# Autodesk Inventor assembly: Counter2
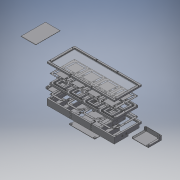
[picture p0: Inventor's stored thumbnail of the model, 180x180]
Saved by Autodesk Inventor 2016 SP2 (Build 200236200, 236)
## iProperties
Created: 2018-06-10
Part Number: Counter2
Material: Generisch
Document SubType Name: Assembly
Designer: Nils
Author: Nils
## Documents named in this file (17)
- C:\Users\Nils\Documents\Inventor\Bastelleien\Counter\Counter2.iam
- C:\Users\Nils\Documents\Inventor\Bastelleien\Counter\Segment_V4.ipt
- C:\Users\Nils\Documents\Inventor\Bastelleien\Counter\Cover_V2.ipt
- C:\Users\Nils\Documents\Inventor\Bastelleien\Counter\Backplate_V2.ipt
- C:\Users\Nils\Documents\Inventor\Bastelleien\Counter\Scheibe.ipt
- C:\Users\Nils\Documents\Inventor\Bastelleien\Counter\Backplate-housing.ipt
- C:\Users\Nils\Documents\Inventor\Bastelleien\Counter\Zwischenplatt.ipt
- C:\Users\Nils\Documents\Inventor\Bastelleien\Counter\Knopf.ipt
- C:\Users\Nils\Documents\Inventor\Bastelleien\Counter\Case-Side.ipt
- C:\Users\Nils\Documents\Inventor\Bastelleien\Counter\Case_side_back.ipt
- C:\Users\Nils\Documents\Inventor\Bastelleien\Counter\Case_bottom_front.ipt
- C:\Users\Nils\Documents\Inventor\Bastelleien\Counter\Case_bottom_back.ipt
- C:\Users\Nils\Documents\Inventor\Bastelleien\Counter\Case_top_back.ipt
- C:\Users\Nils\Documents\Inventor\Bastelleien\Counter\Case-Side_MIR.ipt
- C:\Users\Nils\Documents\Inventor\Bastelleien\Counter\Case_side_back_MIR1.ipt
- C:\Users\Nils\Documents\Inventor\Bastelleien\Counter\Batcap3.ipt
- C:\Users\Nils\Documents\Inventor\Bastelleien\Counter\Batcap3_MIR.ipt
## Components (26 placed, 16 different names)
1. Segment_V4:1 — Passend:3, Passend:4, Fluchtend:1, Fluchtend:2, Fluchtend:3, Passend:11, Fluchtend:4, Fluchtend:5, Fluchtend:6, Fluchtend:26, Fluchtend:27, Passend:34
2. Cover_V2:1 — Passend:3, Fluchtend:7, Fluchtend:8, Fluchtend:9, Passend:14, Fluchtend:10, Fluchtend:11, Fluchtend:12, Passend:21
3. Backplate_V2:1 — Passend:4, Passend:17, Fluchtend:13, Fluchtend:16, Fluchtend:17, Fluchtend:18
4. Segment_V4:2 — Fluchtend:1, Passend:11, Passend:12, Fluchtend:4
5. Cover_V2:2 — Fluchtend:7, Passend:14, Passend:15, Fluchtend:10
6. Backplate_V2:2 — Passend:17, Passend:18, Fluchtend:13, Fluchtend:14, Fluchtend:16, Passend:33
7. Segment_V4:3 — Fluchtend:2, Passend:12, Passend:13, Fluchtend:5
8. Cover_V2:3 — Fluchtend:8, Passend:15, Passend:16, Fluchtend:11
9. Backplate_V2:3 — Passend:18, Passend:19, Fluchtend:14, Fluchtend:15, Fluchtend:17
10. Segment_V4:4 — Fluchtend:3, Passend:13, Fluchtend:6
11. Cover_V2:4 — Fluchtend:9, Passend:16, Fluchtend:12
12. Backplate_V2:4 — Passend:19, Fluchtend:15, Fluchtend:18
13. Scheibe:1 — Fluchtend:26, Fluchtend:27, Passend:21, Passend:31, Passend:32
14. Zwischenplatt:1
15. Knopf:1
16. Case-Side:1 — Fluchtend:28, Fluchtend:29, Fluchtend:33, Passend:23, Fluchtend:35, Fluchtend:36
17. Case_side_back:1 — Fluchtend:28, Fluchtend:29, Fluchtend:32, Fluchtend:34, Passend:22, Passend:23, Fluchtend:40, Passend:32, Passend:33, Passend:34, Fluchtend:45, Fluchtend:46, Fluchtend:48, Fluchtend:49, Passend:36
18. Case_bottom_front:1 — Fluchtend:30, Fluchtend:31, Fluchtend:33, Fluchtend:37, Passend:31
19. Case_bottom_back:1 — Fluchtend:30, Fluchtend:31, Fluchtend:32, Fluchtend:34, Passend:22, Passend:26
20. Backplate-housing:1 — Passend:26, Passend:38, Passend:39
21. Case_bottom_front:2 — Fluchtend:35, Fluchtend:36, Fluchtend:37, Fluchtend:38, Fluchtend:39, Fluchtend:43, Fluchtend:44, Passend:25
22. Case_top_back:1 — Fluchtend:38, Fluchtend:39, Fluchtend:40, Passend:35, Passend:38
23. Case-Side_MIR:1 — Fluchtend:43, Fluchtend:44, Passend:25, Fluchtend:47
24. Case_side_back_MIR1:1 — Fluchtend:45, Fluchtend:46, Passend:35, Fluchtend:47, Fluchtend:50, Fluchtend:51, Passend:37, Passend:39
25. Batcap3:1 — Fluchtend:48, Fluchtend:49, Passend:36
26. Batcap3_MIR:1 — Fluchtend:50, Fluchtend:51, Passend:37
## Relationships (73: Flush 42, Mate 31)
- Passend:3 [Mate] (66.118 mm): Segment_V4:1 ↔ Cover_V2:1
- Passend:4 [Mate] (88.205 mm): Segment_V4:1 ↔ Backplate_V2:1
- [Mate] (66.118 mm): Segment_V4:2 ↔ Cover_V2:2
- [Mate] (88.205 mm): Segment_V4:2 ↔ Backplate_V2:2
- [Mate] (66.118 mm): Segment_V4:3 ↔ Cover_V2:3
- [Mate] (88.205 mm): Segment_V4:3 ↔ Backplate_V2:3
- [Mate] (66.118 mm): Segment_V4:4 ↔ Cover_V2:4
- [Mate] (88.205 mm): Segment_V4:4 ↔ Backplate_V2:4
- Fluchtend:1 [Flush]: Segment_V4:1 ↔ Segment_V4:2
- Fluchtend:2 [Flush]: Segment_V4:1 ↔ Segment_V4:3
- Fluchtend:3 [Flush]: Segment_V4:1 ↔ Segment_V4:4
- Passend:11 [Mate]: Segment_V4:1 ↔ Segment_V4:2
- Passend:12 [Mate]: Segment_V4:2 ↔ Segment_V4:3
- Passend:13 [Mate]: Segment_V4:3 ↔ Segment_V4:4
- Fluchtend:4 [Flush]: Segment_V4:1 ↔ Segment_V4:2
- Fluchtend:5 [Flush]: Segment_V4:1 ↔ Segment_V4:3
- Fluchtend:6 [Flush]: Segment_V4:1 ↔ Segment_V4:4
- Fluchtend:7 [Flush]: Cover_V2:1 ↔ Cover_V2:2
- Fluchtend:8 [Flush]: Cover_V2:1 ↔ Cover_V2:3
- Fluchtend:9 [Flush]: Cover_V2:1 ↔ Cover_V2:4
- Passend:14 [Mate]: Cover_V2:1 ↔ Cover_V2:2
- Passend:15 [Mate]: Cover_V2:2 ↔ Cover_V2:3
- Passend:16 [Mate]: Cover_V2:3 ↔ Cover_V2:4
- Fluchtend:10 [Flush]: Cover_V2:1 ↔ Cover_V2:2
- Fluchtend:11 [Flush]: Cover_V2:1 ↔ Cover_V2:3
- Fluchtend:12 [Flush]: Cover_V2:1 ↔ Cover_V2:4
- Passend:17 [Mate]: Backplate_V2:1 ↔ Backplate_V2:2
- Passend:18 [Mate]: Backplate_V2:2 ↔ Backplate_V2:3
- Passend:19 [Mate]: Backplate_V2:3 ↔ Backplate_V2:4
- Fluchtend:13 [Flush]: Backplate_V2:1 ↔ Backplate_V2:2
- Fluchtend:14 [Flush]: Backplate_V2:2 ↔ Backplate_V2:3
- Fluchtend:15 [Flush]: Backplate_V2:3 ↔ Backplate_V2:4
- Fluchtend:16 [Flush]: Backplate_V2:1 ↔ Backplate_V2:2
- Fluchtend:17 [Flush]: Backplate_V2:1 ↔ Backplate_V2:3
- Fluchtend:18 [Flush]: Backplate_V2:1 ↔ Backplate_V2:4
- Fluchtend:26 [Flush] (0.75 mm): Segment_V4:1 ↔ Scheibe:1
- Fluchtend:27 [Flush] (0.171 mm): Segment_V4:1 ↔ Scheibe:1
- Passend:21 [Mate] (15.632 mm): Cover_V2:1 ↔ Scheibe:1
- Fluchtend:28 [Flush]: Case-Side:1 ↔ Case_side_back:1
- Fluchtend:29 [Flush]: Case-Side:1 ↔ Case_side_back:1
- Fluchtend:30 [Flush]: Case_bottom_front:1 ↔ Case_bottom_back:1
- Fluchtend:31 [Flush]: Case_bottom_front:1 ↔ Case_bottom_back:1
- Fluchtend:32 [Flush]: Case_side_back:1 ↔ Case_bottom_back:1
- Fluchtend:33 [Flush]: Case-Side:1 ↔ Case_bottom_front:1
- Fluchtend:34 [Flush]: Case_side_back:1 ↔ Case_bottom_back:1
- Passend:22 [Mate] (44.139 mm): Case_side_back:1 ↔ Case_bottom_back:1
- Passend:23 [Mate] (68.515 mm): Case-Side:1 ↔ Case_side_back:1
- Fluchtend:35 [Flush]: Case-Side:1 ↔ Case_bottom_front:2
- Fluchtend:36 [Flush]: Case-Side:1 ↔ Case_bottom_front:2
- Fluchtend:37 [Flush]: Case_bottom_front:1 ↔ Case_bottom_front:2
- Fluchtend:38 [Flush]: Case_bottom_front:2 ↔ Case_top_back:1
- Fluchtend:39 [Flush]: Case_bottom_front:2 ↔ Case_top_back:1
- Fluchtend:40 [Flush]: Case_side_back:1 ↔ Case_top_back:1
- Fluchtend:43 [Flush]: Case_bottom_front:2 ↔ Case-Side_MIR:1
- Fluchtend:44 [Flush]: Case_bottom_front:2 ↔ Case-Side_MIR:1
- Passend:25 [Mate] (75.212 mm): Case_bottom_front:2 ↔ Case-Side_MIR:1
- Passend:26 [Mate] (71.173 mm): Case_bottom_back:1 ↔ Backplate-housing:1
- Passend:31 [Mate] (19.515 mm): Scheibe:1 ↔ Case_bottom_front:1
- Passend:32 [Mate]: Scheibe:1 ↔ Case_side_back:1
- Passend:33 [Mate] (31.59 mm): Backplate_V2:2 ↔ Case_side_back:1
- Passend:34 [Mate] (98.618 mm): Segment_V4:1 ↔ Case_side_back:1
- Fluchtend:45 [Flush]: Case_side_back:1 ↔ Case_side_back_MIR1:1
- Fluchtend:46 [Flush]: Case_side_back:1 ↔ Case_side_back_MIR1:1
- Passend:35 [Mate] (44.478 mm): Case_top_back:1 ↔ Case_side_back_MIR1:1
- Fluchtend:47 [Flush]: Case-Side_MIR:1 ↔ Case_side_back_MIR1:1
- Fluchtend:48 [Flush]: Case_side_back:1 ↔ Batcap3:1
- Fluchtend:49 [Flush]: Case_side_back:1 ↔ Batcap3:1
- Passend:36 [Mate] (211.248 mm): Case_side_back:1 ↔ Batcap3:1
- Fluchtend:50 [Flush]: Case_side_back_MIR1:1 ↔ Batcap3_MIR:1
- Fluchtend:51 [Flush]: Case_side_back_MIR1:1 ↔ Batcap3_MIR:1
- Passend:37 [Mate] (270.899 mm): Case_side_back_MIR1:1 ↔ Batcap3_MIR:1
- Passend:38 [Mate]: Backplate-housing:1 ↔ Case_top_back:1
- Passend:39 [Mate]: Backplate-housing:1 ↔ Case_side_back_MIR1:1
## Named parameters: d18_d12 = 66.118 mm, d19_d13 = 50 mm, d20_d14 = 0 mm, d21_d15 = 88.205 mm, d22_d16 = 50 mm, d23_d17 = 0 mm, d24_d12 = 66.118 mm, d25_d13 = 50 mm, d26_d14 = 0 mm, d27_d15 = 88.205 mm, d28_d16 = 50 mm, d29_d17 = 0 mm, d30_d12 = 66.118 mm, d31_d13 = 50 mm, d32_d14 = 0 mm, d33_d15 = 88.205 mm, d34_d16 = 50 mm, d35_d17 = 0 mm
